# Autodesk Inventor assembly: MidSquareFull
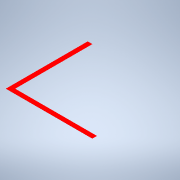
[picture p0: Inventor's stored thumbnail of the model, 180x180]
Saved by Autodesk Inventor 2021 (Build 250183000, 183)
## iProperties
Created: 2021-03-03
Part Number: MidSquareFull
Document SubType Name: Assembly
Designer: CMurray
Author: CMurray
## Documents named in this file (2)
- F:\PHRC CADD 2021\2021 Game Design Challenge\Full Field\Parts\Tape\MidSquareFull.iam
- F:\PHRC CADD 2021\2021 Game Design Challenge\Full Field\Parts\Tape\MidSquareRed1.ipt
## Components (2 placed, 1 different names)
1. MidSquareRed1:1 — Mate:1, Flush:1, Flush:2
2. MidSquareRed1:2 — Mate:1, Flush:1, Flush:2
## Relationships (3: Flush 2, Mate 1)
- Mate:1: MidSquareRed1:1 ↔ MidSquareRed1:2
- Flush:1: MidSquareRed1:1 ↔ MidSquareRed1:2
- Flush:2: MidSquareRed1:1 ↔ MidSquareRed1:2
